# Autodesk Inventor assembly: ArmWithBase
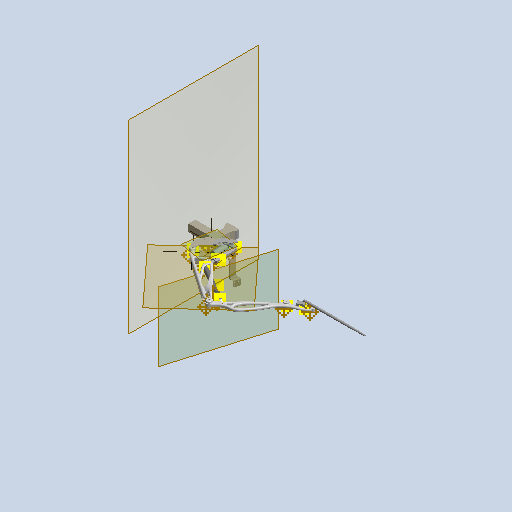
[picture p0: Inventor's stored thumbnail of the model, 512x512]
Saved by Autodesk Inventor 2025.2 (Build 292293000, 293)
## iProperties
Created: 2025-01-19
Part Number: ArmWithBase
Document SubType Name: Assembly
Designer: valer
Author: valer
## Documents named in this file (4)
- D:\str1ker\cad\ArmWithBase.iam
- D:\str1ker\cad\ArmBase.iam
- D:\str1ker\cad\Arm.iam
- D:\str1ker\cad\ScapulaBack.ipt
## Components (3 placed, 3 different names)
1. Base:1 [sub-assembly] — Mate:5, Mate:6, Mate:7, Mate:18, Mate:19, Mate:20, Angle:1
2. Arm:1 [sub-assembly] — Mate:5, Mate:6, Mate:8, Mate:15, Angle:1
3. ScapulaBack:1 — Mate:18, Mate:19, Mate:20
## Relationships (9: Mate 8, Angle 1)
- Mate:5: Base:1 ↔ Arm:1
- Mate:6: Base:1 ↔ Arm:1
- Mate:7: Base:1
- Mate:8: Arm:1
- Mate:15: Arm:1
- Mate:18: Base:1 ↔ ScapulaBack:1
- Mate:19: Base:1 ↔ ScapulaBack:1
- Mate:20: Base:1 ↔ ScapulaBack:1
- Angle:1 (0 deg): Base:1 ↔ Arm:1
